# Autodesk Inventor assembly: Assembly1
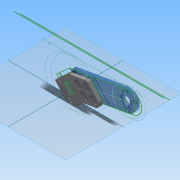
[picture p0: Inventor's stored thumbnail of the model, 180x180]
Saved by Autodesk Inventor 2014 SP2 (Build 180246200, 246)
## iProperties
Created: 2014-05-16
Part Number: Assembly1
Document SubType Name: Assembly
Designer: dliu
Author: dliu
## Documents named in this file (3)
- C:\Users\dliu\Dropbox\dbhome\electric-longboard\dliu\Mount\Mount.iam
- C:\Users\dliu\Dropbox\dbhome\electric-longboard\dliu\Mount\Motor Mount.ipt
- C:\Users\dliu\Dropbox\dbhome\electric-longboard\dliu\Mount\Truck Mount.ipt
## Components (2 placed, 2 different names)
1. Motor Mount:1 — Mate:4, Angle:1, Mate:5
2. Truck Mount:1 — Mate:1, Mate:2, Mate:3, Mate:4, Angle:1, Mate:5
## Relationships (6: Mate 5, Angle 1)
- Mate:1: Truck Mount:1
- Mate:2: Truck Mount:1
- Mate:3: Truck Mount:1
- Mate:4: Motor Mount:1 ↔ Truck Mount:1
- Angle:1 (0 deg): Motor Mount:1 ↔ Truck Mount:1
- Mate:5: Motor Mount:1 ↔ Truck Mount:1
